# Autodesk Inventor assembly: KB33-046-002 - Привод в сборе зеркальный
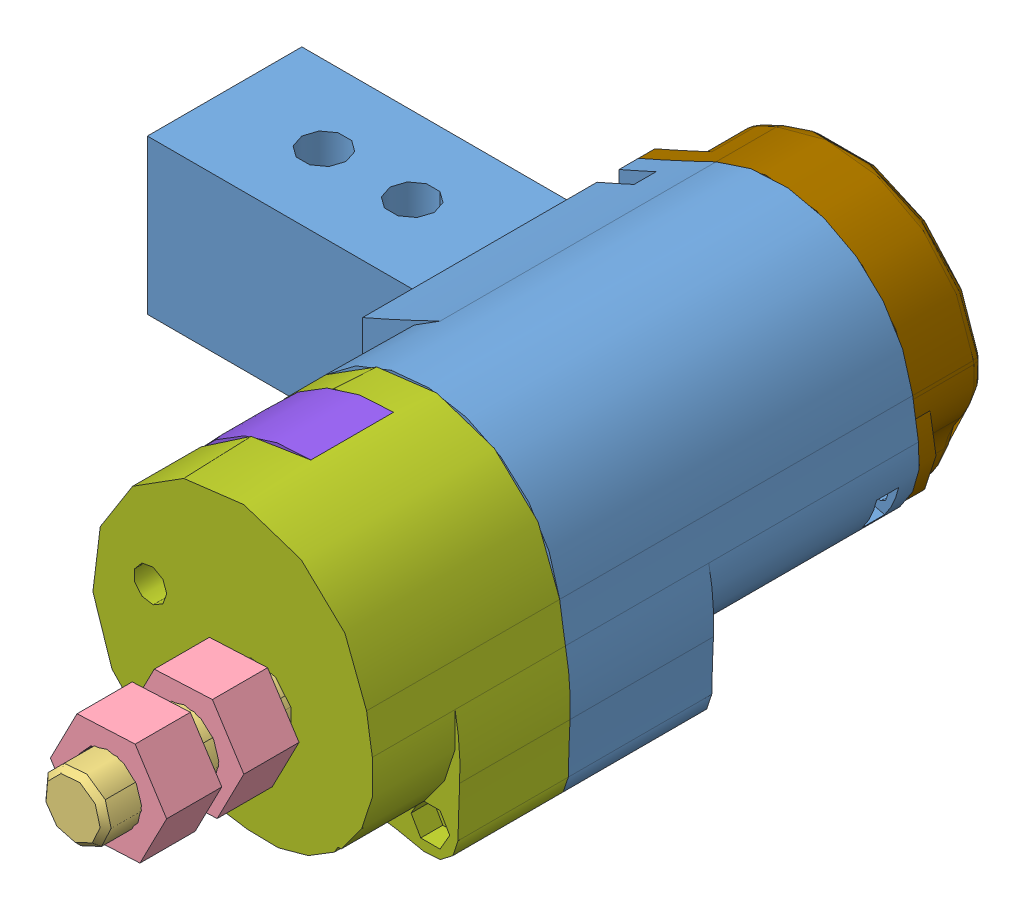
[picture p0: shaded view drawn from the shape stored in the file]
Saved by Autodesk Inventor 2020 (Build 240168000, 168)
## iProperties
Created: 2021-06-21
Part Number: KB33-046-002 - Привод в сборе зеркальный
Document SubType Name: Assembly
Designer: Петров Иван
Mass: 1234.32 g
Surface Area: 1916.85 cm^2
Volume: 1228.12 cm^3
Density: 1.00504 g/cm^3
Author: Петров Иван
## Documents named in this file (11)
- E:\IVAN\Ivan_desktop\Kvantorium\Projects\RoboPatrol\design\KB33-046-002 - Привод в сборе зеркальный.iam
- E:\IVAN\Ivan_desktop\Kvantorium\Projects\RoboPatrol\design\KB33-046-002-001 - Крепление зеркальный.ipt
- E:\IVAN\Ivan_desktop\Kvantorium\Projects\RoboPatrol\design\standart_components\dc_gear_motor_12V_500rpm\dc_gear_motor_12V_500rpm зеркальный1.ipt
- E:\IVAN\Ivan_desktop\Kvantorium\Projects\RoboPatrol\design\standart_components\WheelBig\колесо большое1 зеркальный1.iam
- E:\IVAN\Ivan_desktop\Kvantorium\Projects\RoboPatrol\design\KB33-046-002-002 - Втулка зеркальный.ipt
- E:\IVAN\Ivan_desktop\Kvantorium\Projects\RoboPatrol\design\KB33-046-002-003 - Фиксирующая гайка зеркальный.ipt
- E:\IVAN\Ivan_desktop\Kvantorium\Projects\RoboPatrol\design\KB33-046-002-004 - Колесо энкодера зеркальный.ipt
- E:\IVAN\Ivan_desktop\Kvantorium\Projects\RoboPatrol\design\standart_components\Standart optical endstop зеркальный1.ipt
- E:\IVAN\Ivan_desktop\Kvantorium\Projects\RoboPatrol\design\KB33-046-002-005 - Кожух датчика зеркальный.ipt
- E:\IVAN\Ivan_desktop\Kvantorium\Projects\RoboPatrol\design\KB33-046-002-006 - Заглушка зеркальный.ipt
- E:\IVAN\Ivan_desktop\Kvantorium\Projects\RoboPatrol\design\KB33-046-002-007 - Крышка мотора зеркальный.ipt
## Components (12 placed, 10 different names)
1. KB33-046-002-001 - Крепление зеркальный:1 — Совмещение:2, Совмещение:1, Заподлицо:1, Угол:6, Совмещение:19, Совмещение:17, Совмещение:26, Совмещение:25, Совмещение:24
2. dc_gear_motor_12V_500rpm зеркальный1:1 — Совмещение:2, Совмещение:1, Заподлицо:1, Совмещение:4, Совмещение:3, Угол:1, Совмещение:6, Совмещение:5
3. колесо большое1 зеркальный1:1 [sub-assembly] — Совмещение:4, Совмещение:3, Совмещение:8, Угол:2, Совмещение:10
4. KB33-046-002-002 - Втулка зеркальный:1 — Угол:1, Совмещение:6, Совмещение:5, Совмещение:7, Совмещение:9, Совмещение:12, Угол:3, Совмещение:11, Совмещение:20, Совмещение:16, Совмещение:18
5. KB33-046-002-003 - Фиксирующая гайка зеркальный:1 — Совмещение:8, Угол:2, Совмещение:7, Угол:4
6. KB33-046-002-003 - Фиксирующая гайка зеркальный:2 — Угол:4, Совмещение:10, Совмещение:9
7. KB33-046-002-003 - Фиксирующая гайка зеркальный:3 — Совмещение:12, Угол:3, Совмещение:11, Заподлицо:2, Угол:5
8. KB33-046-002-004 - Колесо энкодера зеркальный:1 — Заподлицо:2, Совмещение:20, Угол:5, Совмещение:15, Касательность:1
9. Standart optical endstop зеркальный1:1 — Совмещение:16, Совмещение:15, Угол:6, Касательность:1, Совмещение:21
10. KB33-046-002-005 - Кожух датчика зеркальный:1 — Совмещение:19, Совмещение:18, Совмещение:17, Совмещение:23, Совмещение:22
11. KB33-046-002-006 - Заглушка зеркальный:1 — Совмещение:23, Совмещение:22, Совмещение:21
12. KB33-046-002-007 - Крышка мотора зеркальный:1 — Совмещение:26, Совмещение:25, Совмещение:24
## Relationships (33: Mate 24, Angle 6, Flush 2, Tangent 1)
- Совмещение:2 [Mate]: KB33-046-002-001 - Крепление зеркальный:1 ↔ dc_gear_motor_12V_500rpm зеркальный1:1
- Совмещение:1 [Mate]: KB33-046-002-001 - Крепление зеркальный:1 ↔ dc_gear_motor_12V_500rpm зеркальный1:1
- Заподлицо:1 [Flush]: KB33-046-002-001 - Крепление зеркальный:1 ↔ dc_gear_motor_12V_500rpm зеркальный1:1
- Совмещение:4 [Mate]: dc_gear_motor_12V_500rpm зеркальный1:1 ↔ колесо большое1 зеркальный1:1
- Совмещение:3 [Mate] (30 mm): dc_gear_motor_12V_500rpm зеркальный1:1 ↔ колесо большое1 зеркальный1:1
- Угол:1 [Angle] (180 deg): dc_gear_motor_12V_500rpm зеркальный1:1 ↔ KB33-046-002-002 - Втулка зеркальный:1
- Совмещение:6 [Mate]: dc_gear_motor_12V_500rpm зеркальный1:1 ↔ KB33-046-002-002 - Втулка зеркальный:1
- Совмещение:5 [Mate]: dc_gear_motor_12V_500rpm зеркальный1:1 ↔ KB33-046-002-002 - Втулка зеркальный:1
- Совмещение:8 [Mate]: колесо большое1 зеркальный1:1 ↔ KB33-046-002-003 - Фиксирующая гайка зеркальный:1
- Угол:2 [Angle] (0 deg): колесо большое1 зеркальный1:1 ↔ KB33-046-002-003 - Фиксирующая гайка зеркальный:1
- Совмещение:7 [Mate]: KB33-046-002-002 - Втулка зеркальный:1 ↔ KB33-046-002-003 - Фиксирующая гайка зеркальный:1
- Угол:4 [Angle] (0 deg): KB33-046-002-003 - Фиксирующая гайка зеркальный:1 ↔ KB33-046-002-003 - Фиксирующая гайка зеркальный:2
- Совмещение:10 [Mate]: колесо большое1 зеркальный1:1 ↔ KB33-046-002-003 - Фиксирующая гайка зеркальный:2
- Совмещение:9 [Mate]: KB33-046-002-002 - Втулка зеркальный:1 ↔ KB33-046-002-003 - Фиксирующая гайка зеркальный:2
- Совмещение:12 [Mate]: KB33-046-002-002 - Втулка зеркальный:1 ↔ KB33-046-002-003 - Фиксирующая гайка зеркальный:3
- Угол:3 [Angle] (0 deg): KB33-046-002-002 - Втулка зеркальный:1 ↔ KB33-046-002-003 - Фиксирующая гайка зеркальный:3
- Совмещение:11 [Mate]: KB33-046-002-002 - Втулка зеркальный:1 ↔ KB33-046-002-003 - Фиксирующая гайка зеркальный:3
- Заподлицо:2 [Flush]: KB33-046-002-003 - Фиксирующая гайка зеркальный:3 ↔ KB33-046-002-004 - Колесо энкодера зеркальный:1
- Совмещение:20 [Mate]: KB33-046-002-002 - Втулка зеркальный:1 ↔ KB33-046-002-004 - Колесо энкодера зеркальный:1
- Угол:5 [Angle] (0 deg): KB33-046-002-003 - Фиксирующая гайка зеркальный:3 ↔ KB33-046-002-004 - Колесо энкодера зеркальный:1
- Совмещение:16 [Mate] (4 mm): KB33-046-002-002 - Втулка зеркальный:1 ↔ Standart optical endstop зеркальный1:1
- Совмещение:15 [Mate] (1 mm): KB33-046-002-004 - Колесо энкодера зеркальный:1 ↔ Standart optical endstop зеркальный1:1
- Угол:6 [Angle] (250 deg): KB33-046-002-001 - Крепление зеркальный:1 ↔ Standart optical endstop зеркальный1:1
- Касательность:1 [Tangent] (2.5 mm): KB33-046-002-004 - Колесо энкодера зеркальный:1 ↔ Standart optical endstop зеркальный1:1
- Совмещение:19 [Mate]: KB33-046-002-001 - Крепление зеркальный:1 ↔ KB33-046-002-005 - Кожух датчика зеркальный:1
- Совмещение:18 [Mate]: KB33-046-002-002 - Втулка зеркальный:1 ↔ KB33-046-002-005 - Кожух датчика зеркальный:1
- Совмещение:17 [Mate]: KB33-046-002-001 - Крепление зеркальный:1 ↔ KB33-046-002-005 - Кожух датчика зеркальный:1
- Совмещение:23 [Mate]: KB33-046-002-005 - Кожух датчика зеркальный:1 ↔ KB33-046-002-006 - Заглушка зеркальный:1
- Совмещение:22 [Mate]: KB33-046-002-005 - Кожух датчика зеркальный:1 ↔ KB33-046-002-006 - Заглушка зеркальный:1
- Совмещение:21 [Mate]: Standart optical endstop зеркальный1:1 ↔ KB33-046-002-006 - Заглушка зеркальный:1
- Совмещение:26 [Mate]: KB33-046-002-001 - Крепление зеркальный:1 ↔ KB33-046-002-007 - Крышка мотора зеркальный:1
- Совмещение:25 [Mate]: KB33-046-002-001 - Крепление зеркальный:1 ↔ KB33-046-002-007 - Крышка мотора зеркальный:1
- Совмещение:24 [Mate]: KB33-046-002-001 - Крепление зеркальный:1 ↔ KB33-046-002-007 - Крышка мотора зеркальный:1
